# Autodesk Inventor assembly: 2nd floor
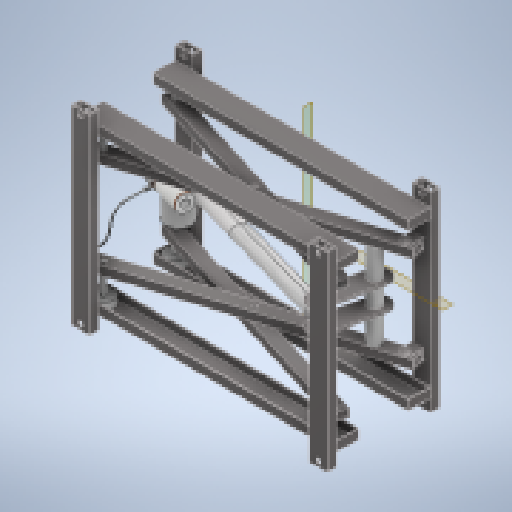
[picture p0: Inventor's stored thumbnail of the model, 512x512]
Saved by Autodesk Inventor 2026.2 (Build 302298010, 298A)
## iProperties
Created: 2026-05-16
Part Number: 2nd floor
Document SubType Name: Assembly
Designer: AdminForWorker
Title: 2nd floor_wheel 고정X v15
Author: AdminForWorker
## Documents named in this file (12)
- C:\Users\chanh\내 드라이브\교과공부\2026년 1학기 (4학년 1학기)\01창의제품설계\CLOSE_hardware\03상체\2nd floor.iam
- C:\Users\chanh\내 드라이브\교과공부\2026년 1학기 (4학년 1학기)\01창의제품설계\CLOSE_hardware\03상체\Bar2 v4.ipt
- C:\Users\chanh\내 드라이브\교과공부\2026년 1학기 (4학년 1학기)\01창의제품설계\CLOSE_hardware\03상체\Bar1 v5.ipt
- C:\Users\chanh\내 드라이브\교과공부\2026년 1학기 (4학년 1학기)\01창의제품설계\CLOSE_hardware\03상체\Bar Bracket v3.ipt
- C:\Users\chanh\내 드라이브\교과공부\2026년 1학기 (4학년 1학기)\01창의제품설계\CLOSE_hardware\03상체\Bar3 v5.ipt
- C:\Users\chanh\내 드라이브\교과공부\2026년 1학기 (4학년 1학기)\01창의제품설계\CLOSE_hardware\03상체\실린더 바 v1.ipt
- C:\Users\chanh\내 드라이브\교과공부\2026년 1학기 (4학년 1학기)\01창의제품설계\CLOSE_hardware\03상체\Linear Motor v5.ipt
- C:\Users\chanh\내 드라이브\교과공부\2026년 1학기 (4학년 1학기)\01창의제품설계\CLOSE_hardware\03상체\Bar Bracket 2 v5.ipt
- C:\Users\chanh\내 드라이브\교과공부\2026년 1학기 (4학년 1학기)\01창의제품설계\CLOSE_hardware\03상체\Linear moter braket v6.ipt
- C:\Users\chanh\내 드라이브\교과공부\2026년 1학기 (4학년 1학기)\01창의제품설계\CLOSE_hardware\03상체\Motor box v4.ipt
- C:\Users\chanh\내 드라이브\교과공부\2026년 1학기 (4학년 1학기)\01창의제품설계\CLOSE_hardware\03상체\wheel_66.ipt
- C:\Users\chanh\내 드라이브\교과공부\2026년 1학기 (4학년 1학기)\01창의제품설계\CLOSE_hardware\03상체\wheel_86.ipt
## Components (26 placed, 11 different names)
1. Bar2 v4:1 — Flush:1, Mate:1, Flush:2, Flush:3, Flush:4, Mate:2, Flush:21, Flush:22, Mate:11, Symmetry:1, Symmetry:2
2. Bar2 v4:2 — Flush:5, Mate:3, Flush:6, Flush:13, Mate:7, Flush:14, Flush:15, Mate:8, Flush:16, Mate:18, Symmetry:1, Symmetry:2
3. Bar1 v5:1 — Flush:1, Mate:1, Flush:2, Tangent:8
4. Bar1 v5:2 — Flush:3, Flush:4, Mate:2, Flush:5, Mate:3, Flush:6, Tangent:9
5. Bar Bracket v9:1 — Flush:13, Mate:7, Flush:14, Rotational:2
6. Bar Bracket v9:2 — Flush:15, Mate:8, Flush:16, Rotational:1
7. Bar3 v5:1 — Rotational:1, Rotational:5, Rigid:2
8. Bar3 v5:2 — Rotational:2, Rotational:6, Rigid:4, Mate:13, Tangent:5, Mate:14, Mate:17
9. Bar3 v5:3 — Rotational:4, Rotational:5, Rigid:1
10. Bar3 v5:4 — Rotational:3, Rotational:6, Rigid:3
11. 실린더 바 v1:1 — Mate:13, Tangent:5, Mate:14, Cylindrical:1
12. Bar2 v4:4 — Flush:7, Mate:4, Flush:8, Flush:9, Mate:5, Flush:10
13. Bar1 v5:3 — Flush:9, Mate:5, Flush:10, Flush:11, Flush:12, Mate:6, Tangent:7
14. Bar1 v5:4 — Flush:7, Mate:4, Flush:8, Tangent:6
15. Bar2 v4:3 — Flush:11, Flush:12, Mate:6, Flush:17, Mate:9, Flush:18, Flush:19, Mate:10, Flush:20, Mate:18
16. Bar Bracket v9:3 — Flush:17, Mate:9, Flush:18, Rotational:4
17. Bar Bracket v9:4 — Flush:19, Mate:10, Flush:20, Rotational:3
18. Linear Motor v5:1 — Rotational:7, Tangent:12, Mate:19, Tangent:13
19. Bar Bracket 2 v5:1 — Rotational:7, Flush:21, Flush:22, Mate:11
20. Linear moter braket v6:1 — Flush:23, Flush:24, Mate:15, Mate:17
21. Linear moter braket v6:2 — Flush:23, Flush:24, Mate:15, Cylindrical:1
22. Motor box v4:1 — Tangent:12, Mate:19, Tangent:13
23. wheel_66:1 — Rigid:1, Tangent:8
24. wheel_86:1 — Rigid:2, Tangent:7
25. wheel_66:2 — Rigid:3, Tangent:9
26. wheel_86:2 — Rigid:4, Tangent:6
## Relationships (62: Flush 24, Mate 17, RevoluteJoint 7, Tangent 7, WeldJoint 4, Symmetry 2, CylindricalJoint 1)
- Flush:1 (30 mm): Bar2 v4:1 ↔ Bar1 v5:1
- Mate:1: Bar2 v4:1 ↔ Bar1 v5:1
- Flush:2: Bar2 v4:1 ↔ Bar1 v5:1
- Flush:3 (30 mm): Bar2 v4:1 ↔ Bar1 v5:2
- Flush:4: Bar2 v4:1 ↔ Bar1 v5:2
- Mate:2: Bar2 v4:1 ↔ Bar1 v5:2
- Flush:5: Bar2 v4:2 ↔ Bar1 v5:2
- Mate:3: Bar2 v4:2 ↔ Bar1 v5:2
- Flush:6 (30 mm): Bar2 v4:2 ↔ Bar1 v5:2
- Flush:7 (30 mm): Bar2 v4:4 ↔ Bar1 v5:4
- Mate:4: Bar2 v4:4 ↔ Bar1 v5:4
- Flush:8: Bar2 v4:4 ↔ Bar1 v5:4
- Flush:9 (30 mm): Bar2 v4:4 ↔ Bar1 v5:3
- Mate:5: Bar2 v4:4 ↔ Bar1 v5:3
- Flush:10: Bar2 v4:4 ↔ Bar1 v5:3
- Flush:11 (30 mm): Bar1 v5:3 ↔ Bar2 v4:3
- Flush:12: Bar1 v5:3 ↔ Bar2 v4:3
- Mate:6: Bar1 v5:3 ↔ Bar2 v4:3
- Flush:13: Bar2 v4:2 ↔ Bar Bracket v9:1
- Mate:7 (-8 mm): Bar2 v4:2 ↔ Bar Bracket v9:1
- Flush:14 (96 mm): Bar2 v4:2 ↔ Bar Bracket v9:1
- Flush:15 (96 mm): Bar2 v4:2 ↔ Bar Bracket v9:2
- Mate:8 (-8 mm): Bar2 v4:2 ↔ Bar Bracket v9:2
- Flush:16: Bar2 v4:2 ↔ Bar Bracket v9:2
- Flush:17 (76 mm): Bar2 v4:3 ↔ Bar Bracket v9:3
- Mate:9 (-8 mm): Bar2 v4:3 ↔ Bar Bracket v9:3
- Flush:18: Bar2 v4:3 ↔ Bar Bracket v9:3
- Flush:19: Bar2 v4:3 ↔ Bar Bracket v9:4
- Mate:10 (-8 mm): Bar2 v4:3 ↔ Bar Bracket v9:4
- Flush:20 (76 mm): Bar2 v4:3 ↔ Bar Bracket v9:4
- Rotational:1 [RevoluteJoint]: Bar Bracket v9:2 ↔ Bar3 v5:1
- Rotational:2 [RevoluteJoint]: Bar Bracket v9:1 ↔ Bar3 v5:2
- Rotational:3 [RevoluteJoint]: Bar3 v5:4 ↔ Bar Bracket v9:4
- Rotational:4 [RevoluteJoint]: Bar3 v5:3 ↔ Bar Bracket v9:3
- Rotational:5 [RevoluteJoint]: Bar3 v5:1 ↔ Bar3 v5:3
- Rotational:6 [RevoluteJoint]: Bar3 v5:2 ↔ Bar3 v5:4
- Rotational:7 [RevoluteJoint]: Linear Motor v5:1 ↔ Bar Bracket 2 v5:1
- Flush:21 (208.5 mm): Bar2 v4:1 ↔ Bar Bracket 2 v5:1
- Flush:22: Bar2 v4:1 ↔ Bar Bracket 2 v5:1
- Mate:11: Bar2 v4:1 ↔ Bar Bracket 2 v5:1
- Rigid:1 [WeldJoint]: Bar3 v5:3 ↔ wheel_66:1
- Rigid:2 [WeldJoint]: Bar3 v5:1 ↔ wheel_86:1
- Rigid:3 [WeldJoint]: Bar3 v5:4 ↔ wheel_66:2
- Rigid:4 [WeldJoint]: Bar3 v5:2 ↔ wheel_86:2
- Mate:13 (-80 mm): Bar3 v5:2 ↔ 실린더 바 v1:1
- Tangent:5: Bar3 v5:2 ↔ 실린더 바 v1:1
- Mate:14: Bar3 v5:2 ↔ 실린더 바 v1:1
- Flush:23 (55 mm): Linear moter braket v6:1 ↔ Linear moter braket v6:2
- Flush:24: Linear moter braket v6:1 ↔ Linear moter braket v6:2
- Mate:15: Linear moter braket v6:1 ↔ Linear moter braket v6:2
- Mate:17 (71 mm): Bar3 v5:2 ↔ Linear moter braket v6:1
- Tangent:6: Bar1 v5:4 ↔ wheel_86:2
- Tangent:7: Bar1 v5:3 ↔ wheel_86:1
- Tangent:8: Bar1 v5:1 ↔ wheel_66:1
- Tangent:9: Bar1 v5:2 ↔ wheel_66:2
- Mate:18 (-260 mm): Bar2 v4:2 ↔ Bar2 v4:3
- Tangent:12: Linear Motor v5:1 ↔ Motor box v4:1
- Mate:19: Linear Motor v5:1 ↔ Motor box v4:1
- Tangent:13: Linear Motor v5:1 ↔ Motor box v4:1
- Cylindrical:1: 실린더 바 v1:1 ↔ Linear moter braket v6:2
- Symmetry:1: Bar2 v4:1 ↔ Bar2 v4:2
- Symmetry:2: Bar2 v4:1 ↔ Bar2 v4:2
